# Autodesk Inventor assembly: SlaveBot
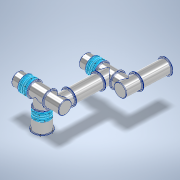
[picture p0: Inventor's stored thumbnail of the model, 180x180]
Saved by Autodesk Inventor 2021 (Build 250183000, 183)
## iProperties
Created: 2020-05-10
Part Number: SlaveBot
Document SubType Name: Assembly
Designer: avi41
Author: avi41
## Documents named in this file (21)
- C:\Users\avi41\Desktop\Robot Arm\CAD_files\SlaveBot.iam
- C:\Users\avi41\Desktop\Robot Arm\CAD_files\Base.ipt
- C:\Users\avi41\Desktop\Robot Arm\CAD_files\Link_1.ipt
- C:\Users\avi41\Desktop\Robot Arm\CAD_files\Joint_0_1.iam
- C:\Users\avi41\Documents\Inventor\Content Center Files\R2020\en-US\ISO 8738(1)\ISO 8738 - 4(1).ipt
- C:\Users\avi41\Documents\Inventor\Content Center Files\R2020\en-US\ANSI B18.3.4M(2)\ANSI B18.3.4M - M5 x 0.8 x 20(1).ipt
- C:\Users\avi41\Documents\Inventor\Content Center Files\R2020\en-US\ANSI B18.3.4M(2)\ANSI B18.3.4M - M4 x 0.7 x 25(1).ipt
- C:\Users\avi41\Desktop\Robot Arm\CAD_files\Joint_1_2.iam
- C:\Users\avi41\Desktop\Robot Arm\CAD_files\Cover_Joint_1_2.ipt
- C:\Users\avi41\Desktop\Robot Arm\CAD_files\MCOCWK26-6-12.iam
- C:\Users\avi41\Desktop\Robot Arm\CAD_files\PRT_01_30_H1_1.iam
- C:\Users\avi41\Desktop\Robot Arm\CAD_files\Adapter_bearing_joint.ipt
- C:\Users\avi41\Desktop\Robot Arm\CAD_files\Adapter_bearing_link.ipt
- C:\Users\avi41\Desktop\Robot Arm\CAD_files\Link_1_b.ipt
- C:\Users\avi41\Desktop\Robot Arm\CAD_files\Connection_link_1.ipt
- C:\Users\avi41\Desktop\Robot Arm\CAD_files\Link_2.ipt
- C:\Users\avi41\Desktop\Robot Arm\CAD_files\Joint_2_3.iam
- C:\Users\avi41\Desktop\Robot Arm\CAD_files\Cover_Joint_2_3.ipt
- C:\Users\avi41\Desktop\Robot Arm\CAD_files\Connection_link_2.ipt
- C:\Users\avi41\Desktop\Robot Arm\CAD_files\Link_2_b.ipt
- C:\Users\avi41\Desktop\Robot Arm\CAD_files\Link_3.ipt
## Components (48 placed, 20 different names)
1. Base:1 — Flush:1, Flush:2, Mate:1, Insert:1, Insert:2, Insert:3, Insert:4, Insert:5, Mate:38, Mate:39, Mate:40
2. Link_1:1 — Mate:29, Mate:30, Mate:31, Mate:53, Mate:54, Mate:55
3. Joint_1_2:1 [sub-assembly] — Mate:29, Mate:30, Mate:31, Mate:35, Mate:36, Mate:37, Mate:58, Angle:2, Mate:59, Mate:70, Mate:71, Mate:72
4. Cover_Joint_1_2:1 — Mate:35, Mate:36, Mate:37
5. Joint_0_1:1 [sub-assembly] — Mate:38, Mate:39, Mate:40, Mate:41, Mate:42, Mate:43, Mate:44, Mate:45, Mate:46, Mate:47, Mate:48, Mate:49, Mate:50, Mate:51, Mate:52, Mate:53, Mate:54, Mate:55, Mate:56, Angle:1, Mate:57, Mate:61, Mate:62, Mate:63
6. MCOCWK26-6-12:1 [sub-assembly] — Mate:56, Angle:1, Mate:57, Mate:60, Mate:66
7. MCOCWK26-6-12:2 [sub-assembly] — Mate:58, Angle:2, Mate:59, Mate:76
8. PRT_01_30_H1_1:1 [sub-assembly] — Mate:60, Mate:64, Mate:65, Mate:67, Mate:68
9. Adapter_bearing_joint:1 — Mate:61, Mate:62, Mate:63, Mate:64, Mate:65
10. Adapter_bearing_link:1 — Mate:66, Mate:67, Mate:68
11. Link_1_b:1 — Mate:82, Mate:83, Mate:84, Mate:85, Mate:86, Mate:87
12. PRT_01_30_H1_1:2 [sub-assembly] — Mate:73, Mate:74, Mate:75, Mate:77, Mate:78
13. Adapter_bearing_joint:2 — Mate:70, Mate:71, Mate:72, Mate:73, Mate:74, Mate:75
14. Adapter_bearing_link:2 — Mate:76, Mate:77, Mate:78, Mate:79, Mate:80, Mate:81
15. Connection_link_1:1 — Mate:79, Mate:80, Mate:81, Mate:82, Mate:83, Mate:84
16. Link_2:1 — Mate:85, Mate:86, Mate:87, Mate:88, Mate:89, Mate:90
17. Link_1:2 — Mate:88, Mate:89, Mate:90, Mate:91, Mate:92, Mate:93
18. Joint_2_3:1 [sub-assembly] — Mate:91, Mate:92, Mate:93, Mate:94, Mate:95, Mate:96, Mate:97, Mate:98, Mate:99, Mate:100, Mate:101
19. Cover_Joint_2_3:1 — Mate:94, Mate:95, Mate:96
20. MCOCWK26-6-12:3 [sub-assembly] — Mate:97, Mate:98, Mate:105
21. PRT_01_30_H1_1:3 [sub-assembly] — Mate:102, Mate:103, Mate:104, Mate:106, Mate:107, Mate:108
22. Connection_link_2:1 — Mate:109, Mate:110, Mate:111, Mate:112, Mate:113, Mate:114
23. Adapter_bearing_joint:3 — Mate:99, Mate:100, Mate:101, Mate:102, Mate:103, Mate:104
24. Adapter_bearing_link:3 — Mate:105, Mate:106, Mate:107, Mate:108, Mate:109, Mate:110, Mate:111
25. Link_2_b:1 — Mate:112, Mate:113, Mate:114, Mate:115, Mate:116, Mate:117
26. Link_3:1 — Mate:115, Mate:116, Mate:117
27. DIN EN 28738 4:6 — Mate:17, Mate:18, Mate:42
28. DIN EN 28738 4:7 — Mate:23, Mate:24, Mate:44
29. DIN EN 28738 4:8 — Mate:19, Mate:20, Mate:52
30. DIN EN 28738 4:9 — Mate:21, Mate:22, Mate:50
31. DIN EN 28738 4:10 — Mate:25, Mate:26, Mate:48
32. DIN EN 28738 4:11 — Mate:27, Mate:28, Mate:46
33. Forged Hexagon Socket Button Head Cap Screw - Metric M4 x 0.7 x 25:1 — Mate:19, Mate:20, Mate:51
34. Forged Hexagon Socket Button Head Cap Screw - Metric M4 x 0.7 x 25:2 — Mate:21, Mate:22, Mate:49
35. Forged Hexagon Socket Button Head Cap Screw - Metric M4 x 0.7 x 25:3 — Mate:23, Mate:24, Mate:43
36. Forged Hexagon Socket Button Head Cap Screw - Metric M4 x 0.7 x 25:4 — Mate:25, Mate:26, Mate:47
37. Forged Hexagon Socket Button Head Cap Screw - Metric M4 x 0.7 x 25:5 — Mate:27, Mate:28, Mate:45
38. Forged Hexagon Socket Button Head Cap Screw - Metric M4 x 0.7 x 25:6 — Mate:17, Mate:18, Mate:41
39. DIN EN 28738 4:1 — Insert:1, Mate:7, Mate:16
40. DIN EN 28738 4:2 — Insert:2, Mate:10, Mate:15
41. DIN EN 28738 4:3 — Insert:3, Mate:11, Mate:14
42. DIN EN 28738 4:4 — Insert:4, Mate:9, Mate:13
43. DIN EN 28738 4:5 — Insert:5, Mate:8, Mate:12
44. Forged Hexagon Socket Button Head Cap Screw - Metric M5 x 0.8 x 20:1 — Mate:7, Mate:16
45. Forged Hexagon Socket Button Head Cap Screw - Metric M5 x 0.8 x 20:2 — Mate:8, Mate:12
46. Forged Hexagon Socket Button Head Cap Screw - Metric M5 x 0.8 x 20:3 — Mate:9, Mate:13
47. Forged Hexagon Socket Button Head Cap Screw - Metric M5 x 0.8 x 20:4 — Mate:11, Mate:14
48. Forged Hexagon Socket Button Head Cap Screw - Metric M5 x 0.8 x 20:5 — Mate:10, Mate:15
## Relationships (117: Mate 108, Insert 5, Flush 2, Angle 2)
- Flush:1: Base:1
- Flush:2: Base:1
- Mate:1: Base:1
- Insert:1: Base:1 ↔ DIN EN 28738 4:1
- Insert:2: Base:1 ↔ DIN EN 28738 4:2
- Insert:3: Base:1 ↔ DIN EN 28738 4:3
- Insert:4: Base:1 ↔ DIN EN 28738 4:4
- Insert:5: Base:1 ↔ DIN EN 28738 4:5
- Mate:7: DIN EN 28738 4:1 ↔ Forged Hexagon Socket Button Head Cap Screw - Metric M5 x 0.8 x 20:1
- Mate:8: DIN EN 28738 4:5 ↔ Forged Hexagon Socket Button Head Cap Screw - Metric M5 x 0.8 x 20:2
- Mate:9: DIN EN 28738 4:4 ↔ Forged Hexagon Socket Button Head Cap Screw - Metric M5 x 0.8 x 20:3
- Mate:10: DIN EN 28738 4:2 ↔ Forged Hexagon Socket Button Head Cap Screw - Metric M5 x 0.8 x 20:5
- Mate:11: DIN EN 28738 4:3 ↔ Forged Hexagon Socket Button Head Cap Screw - Metric M5 x 0.8 x 20:4
- Mate:12: DIN EN 28738 4:5 ↔ Forged Hexagon Socket Button Head Cap Screw - Metric M5 x 0.8 x 20:2
- Mate:13: DIN EN 28738 4:4 ↔ Forged Hexagon Socket Button Head Cap Screw - Metric M5 x 0.8 x 20:3
- Mate:14: DIN EN 28738 4:3 ↔ Forged Hexagon Socket Button Head Cap Screw - Metric M5 x 0.8 x 20:4
- Mate:15: DIN EN 28738 4:2 ↔ Forged Hexagon Socket Button Head Cap Screw - Metric M5 x 0.8 x 20:5
- Mate:16: DIN EN 28738 4:1 ↔ Forged Hexagon Socket Button Head Cap Screw - Metric M5 x 0.8 x 20:1
- Mate:17: DIN EN 28738 4:6 ↔ Forged Hexagon Socket Button Head Cap Screw - Metric M4 x 0.7 x 25:6
- Mate:18: DIN EN 28738 4:6 ↔ Forged Hexagon Socket Button Head Cap Screw - Metric M4 x 0.7 x 25:6
- Mate:19: DIN EN 28738 4:8 ↔ Forged Hexagon Socket Button Head Cap Screw - Metric M4 x 0.7 x 25:1
- Mate:20: DIN EN 28738 4:8 ↔ Forged Hexagon Socket Button Head Cap Screw - Metric M4 x 0.7 x 25:1
- Mate:21: DIN EN 28738 4:9 ↔ Forged Hexagon Socket Button Head Cap Screw - Metric M4 x 0.7 x 25:2
- Mate:22: DIN EN 28738 4:9 ↔ Forged Hexagon Socket Button Head Cap Screw - Metric M4 x 0.7 x 25:2
- Mate:23: DIN EN 28738 4:7 ↔ Forged Hexagon Socket Button Head Cap Screw - Metric M4 x 0.7 x 25:3
- Mate:24: DIN EN 28738 4:7 ↔ Forged Hexagon Socket Button Head Cap Screw - Metric M4 x 0.7 x 25:3
- Mate:25: DIN EN 28738 4:10 ↔ Forged Hexagon Socket Button Head Cap Screw - Metric M4 x 0.7 x 25:4
- Mate:26: DIN EN 28738 4:10 ↔ Forged Hexagon Socket Button Head Cap Screw - Metric M4 x 0.7 x 25:4
- Mate:27: DIN EN 28738 4:11 ↔ Forged Hexagon Socket Button Head Cap Screw - Metric M4 x 0.7 x 25:5
- Mate:28: DIN EN 28738 4:11 ↔ Forged Hexagon Socket Button Head Cap Screw - Metric M4 x 0.7 x 25:5
- Mate:29: Link_1:1 ↔ Joint_1_2:1
- Mate:30: Link_1:1 ↔ Joint_1_2:1
- Mate:31: Link_1:1 ↔ Joint_1_2:1
- Mate:35: Joint_1_2:1 ↔ Cover_Joint_1_2:1
- Mate:36: Joint_1_2:1 ↔ Cover_Joint_1_2:1
- Mate:37: Joint_1_2:1 ↔ Cover_Joint_1_2:1
- Mate:38: Base:1 ↔ Joint_0_1:1
- Mate:39: Base:1 ↔ Joint_0_1:1
- Mate:40: Base:1 ↔ Joint_0_1:1
- Mate:41: Joint_0_1:1 ↔ Forged Hexagon Socket Button Head Cap Screw - Metric M4 x 0.7 x 25:6
- Mate:42: Joint_0_1:1 ↔ DIN EN 28738 4:6
- Mate:43: Joint_0_1:1 ↔ Forged Hexagon Socket Button Head Cap Screw - Metric M4 x 0.7 x 25:3
- Mate:44: Joint_0_1:1 ↔ DIN EN 28738 4:7
- Mate:45: Joint_0_1:1 ↔ Forged Hexagon Socket Button Head Cap Screw - Metric M4 x 0.7 x 25:5
- Mate:46: Joint_0_1:1 ↔ DIN EN 28738 4:11
- Mate:47: Joint_0_1:1 ↔ Forged Hexagon Socket Button Head Cap Screw - Metric M4 x 0.7 x 25:4
- Mate:48: Joint_0_1:1 ↔ DIN EN 28738 4:10
- Mate:49: Joint_0_1:1 ↔ Forged Hexagon Socket Button Head Cap Screw - Metric M4 x 0.7 x 25:2
- Mate:50: Joint_0_1:1 ↔ DIN EN 28738 4:9
- Mate:51: Joint_0_1:1 ↔ Forged Hexagon Socket Button Head Cap Screw - Metric M4 x 0.7 x 25:1
- Mate:52: Joint_0_1:1 ↔ DIN EN 28738 4:8
- Mate:53: Link_1:1 ↔ Joint_0_1:1
- Mate:54: Link_1:1 ↔ Joint_0_1:1
- Mate:55: Link_1:1 ↔ Joint_0_1:1
- Mate:56: Joint_0_1:1 ↔ MCOCWK26-6-12:1
- Angle:1 (0 deg): Joint_0_1:1 ↔ MCOCWK26-6-12:1
- Mate:57 (1.5 mm): Joint_0_1:1 ↔ MCOCWK26-6-12:1
- Mate:58: Joint_1_2:1 ↔ MCOCWK26-6-12:2
- Angle:2 (0 deg): Joint_1_2:1 ↔ MCOCWK26-6-12:2
- Mate:59 (1.5 mm): Joint_1_2:1 ↔ MCOCWK26-6-12:2
- Mate:60: MCOCWK26-6-12:1 ↔ PRT_01_30_H1_1:1
- Mate:61: Joint_0_1:1 ↔ Adapter_bearing_joint:1
- Mate:62: Joint_0_1:1 ↔ Adapter_bearing_joint:1
- Mate:63: Joint_0_1:1 ↔ Adapter_bearing_joint:1
- Mate:64: PRT_01_30_H1_1:1 ↔ Adapter_bearing_joint:1
- Mate:65: PRT_01_30_H1_1:1 ↔ Adapter_bearing_joint:1
- Mate:66: MCOCWK26-6-12:1 ↔ Adapter_bearing_link:1
- Mate:67: PRT_01_30_H1_1:1 ↔ Adapter_bearing_link:1
- Mate:68: PRT_01_30_H1_1:1 ↔ Adapter_bearing_link:1
- Mate:70: Joint_1_2:1 ↔ Adapter_bearing_joint:2
- Mate:71: Joint_1_2:1 ↔ Adapter_bearing_joint:2
- Mate:72: Joint_1_2:1 ↔ Adapter_bearing_joint:2
- Mate:73: PRT_01_30_H1_1:2 ↔ Adapter_bearing_joint:2
- Mate:74: PRT_01_30_H1_1:2 ↔ Adapter_bearing_joint:2
- Mate:75: PRT_01_30_H1_1:2 ↔ Adapter_bearing_joint:2
- Mate:76: MCOCWK26-6-12:2 ↔ Adapter_bearing_link:2
- Mate:77: PRT_01_30_H1_1:2 ↔ Adapter_bearing_link:2
- Mate:78: PRT_01_30_H1_1:2 ↔ Adapter_bearing_link:2
- Mate:79: Adapter_bearing_link:2 ↔ Connection_link_1:1
- Mate:80: Adapter_bearing_link:2 ↔ Connection_link_1:1
- Mate:81: Adapter_bearing_link:2 ↔ Connection_link_1:1
- Mate:82: Link_1_b:1 ↔ Connection_link_1:1
- Mate:83: Link_1_b:1 ↔ Connection_link_1:1
- Mate:84: Link_1_b:1 ↔ Connection_link_1:1
- Mate:85: Link_1_b:1 ↔ Link_2:1
- Mate:86: Link_1_b:1 ↔ Link_2:1
- Mate:87: Link_1_b:1 ↔ Link_2:1
- Mate:88: Link_2:1 ↔ Link_1:2
- Mate:89: Link_2:1 ↔ Link_1:2
- Mate:90: Link_2:1 ↔ Link_1:2
- Mate:91: Link_1:2 ↔ Joint_2_3:1
- Mate:92: Link_1:2 ↔ Joint_2_3:1
- Mate:93: Link_1:2 ↔ Joint_2_3:1
- Mate:94: Joint_2_3:1 ↔ Cover_Joint_2_3:1
- Mate:95: Joint_2_3:1 ↔ Cover_Joint_2_3:1
- Mate:96: Joint_2_3:1 ↔ Cover_Joint_2_3:1
- Mate:97: Joint_2_3:1 ↔ MCOCWK26-6-12:3
- Mate:98 (0.5 mm): Joint_2_3:1 ↔ MCOCWK26-6-12:3
- Mate:99: Joint_2_3:1 ↔ Adapter_bearing_joint:3
- Mate:100: Joint_2_3:1 ↔ Adapter_bearing_joint:3
- Mate:101: Joint_2_3:1 ↔ Adapter_bearing_joint:3
- Mate:102: PRT_01_30_H1_1:3 ↔ Adapter_bearing_joint:3
- Mate:103: PRT_01_30_H1_1:3 ↔ Adapter_bearing_joint:3
- Mate:104: PRT_01_30_H1_1:3 ↔ Adapter_bearing_joint:3
- Mate:105: MCOCWK26-6-12:3 ↔ Adapter_bearing_link:3
- Mate:106: PRT_01_30_H1_1:3 ↔ Adapter_bearing_link:3
- Mate:107: PRT_01_30_H1_1:3 ↔ Adapter_bearing_link:3
- Mate:108: PRT_01_30_H1_1:3 ↔ Adapter_bearing_link:3
- Mate:109: Connection_link_2:1 ↔ Adapter_bearing_link:3
- Mate:110: Connection_link_2:1 ↔ Adapter_bearing_link:3
- Mate:111: Connection_link_2:1 ↔ Adapter_bearing_link:3
- Mate:112: Connection_link_2:1 ↔ Link_2_b:1
- Mate:113: Connection_link_2:1 ↔ Link_2_b:1
- Mate:114: Connection_link_2:1 ↔ Link_2_b:1
- Mate:115: Link_2_b:1 ↔ Link_3:1
- Mate:116: Link_2_b:1 ↔ Link_3:1
- Mate:117: Link_2_b:1 ↔ Link_3:1
